# Autodesk Inventor assembly: all_body
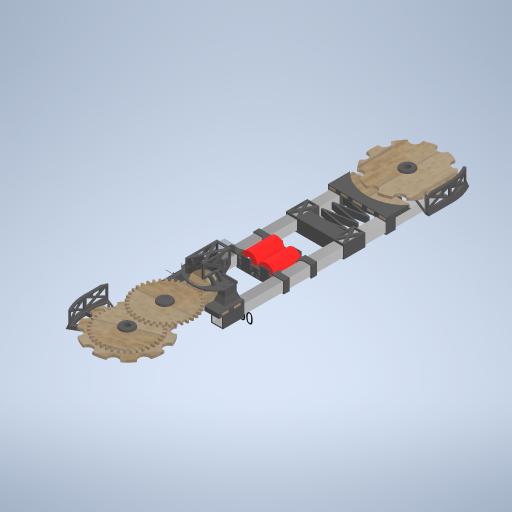
[picture p0: Inventor's stored thumbnail of the model, 512x512]
Saved by Autodesk Inventor 2024.1 (Build 281209000, 209)
## iProperties
Created: 2024-11-06
Part Number: all_body
Document SubType Name: Assembly
Designer: hibik
Author: hibik
## Documents named in this file (8)
- C:\Users\hibik\Documents\Robomech\conveyer\all_body.iam
- C:\Users\hibik\Documents\Robomech\conveyer\ギアボックス.iam
- C:\Users\hibik\Documents\Robomech\conveyer\ギアプレート.iam
- C:\Users\hibik\Documents\Robomech\conveyer\bar_long.ipt
- C:\Users\hibik\Documents\Robomech\conveyer\spring.ipt
- C:\Users\hibik\Documents\Robomech\conveyer\ギア受け_ダンパ.ipt
- C:\Users\hibik\Documents\Robomech\conveyer\電池ボックス.ipt
- C:\Users\hibik\Documents\Robomech\conveyer\電池.ipt
## Components (9 placed, 7 different names)
1. ギアボックス:1 [sub-assembly] — フラッシュ:1, フラッシュ:2, 挿入:1, 挿入:2, 挿入:3, 挿入:4
2. ギアプレート:1 [sub-assembly] — フラッシュ:1, フラッシュ:2
3. bar_long:1 — 挿入:1, 挿入:2, 挿入:5, 挿入:6
4. bar_long:2 — 挿入:3, 挿入:4, メイト:24, メイト:25
5. spring:1 — メイト:1, メイト:2, メイト:3
6. ギア受け_ダンパ:1 — 挿入:5, 挿入:6, メイト:1, メイト:2, メイト:3
7. 電池ボックス:1 — メイト:24, メイト:25, 挿入:7, 挿入:8
8. 電池:1 — 挿入:7
9. 電池:2 — 挿入:8
## Relationships (15: Insert 8, Mate 5, Flush 2)
- フラッシュ:1 [Flush]: ギアボックス:1 ↔ ギアプレート:1
- フラッシュ:2 [Flush]: ギアボックス:1 ↔ ギアプレート:1
- 挿入:1 [Insert]: ギアボックス:1 ↔ bar_long:1
- 挿入:2 [Insert]: ギアボックス:1 ↔ bar_long:1
- 挿入:3 [Insert]: ギアボックス:1 ↔ bar_long:2
- 挿入:4 [Insert]: ギアボックス:1 ↔ bar_long:2
- 挿入:5 [Insert]: bar_long:1 ↔ ギア受け_ダンパ:1
- 挿入:6 [Insert]: bar_long:1 ↔ ギア受け_ダンパ:1
- メイト:1 [Mate]: spring:1 ↔ ギア受け_ダンパ:1
- メイト:2 [Mate]: spring:1 ↔ ギア受け_ダンパ:1
- メイト:3 [Mate] (1 mm): spring:1 ↔ ギア受け_ダンパ:1
- メイト:24 [Mate]: bar_long:2 ↔ 電池ボックス:1
- メイト:25 [Mate]: bar_long:2 ↔ 電池ボックス:1
- 挿入:7 [Insert]: 電池ボックス:1 ↔ 電池:1
- 挿入:8 [Insert]: 電池ボックス:1 ↔ 電池:2
